# Autodesk Inventor assembly: Сборка
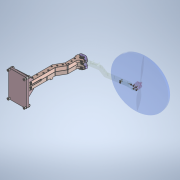
[picture p0: Inventor's stored thumbnail of the model, 180x180]
Saved by Autodesk Inventor 2021.2 (Build 252289000, 289)
## iProperties
Created: 2024-10-29
Part Number: Сборка
Document SubType Name: Assembly
Designer: barko
Mass: 1383.59 g
Surface Area: 2828.64 cm^2
Volume: 1218.78 cm^3
Density: 1.13522 g/cm^3
Author: barko
## Documents named in this file (33)
- C:\Users\DELL\Desktop\Personal\PID_controller\PID_controller\Mechanics\3D_model\Сборка.iam
- C:\Users\DELL\Desktop\Personal\PID_controller\PID_controller\Mechanics\3D_model\Детали твёрдого тела\Скобка 1.ipt
- C:\Users\DELL\Desktop\Personal\PID_controller\PID_controller\Mechanics\3D_model\Детали твёрдого тела\Скобка 2.ipt
- C:\Users\DELL\Desktop\Personal\PID_controller\PID_controller\Mechanics\3D_model\Детали твёрдого тела\Фланец.ipt
- C:\Users\DELL\Desktop\Personal\PID_controller\PID_controller\Mechanics\3D_model\Детали твёрдого тела\Луч.ipt
- C:\Users\DELL\Desktop\Personal\PID_controller\PID_controller\Mechanics\3D_model\Детали твёрдого тела\Ложечка.ipt
- C:\Users\DELL\Desktop\Personal\PID_controller\PID_controller\Mechanics\3D_model\Моторчик.ipt
- C:\Users\DELL\Desktop\Personal\PID_controller\PID_controller\Mechanics\3D_model\Пропеллер.ipt
- C:\Users\DELL\Documents\Inventor\Content Center Files\R2021\ru-RU\Nut GOST 15524-70\Гайка M4-6H ГОСТ 15524-70.ipt
- C:\Users\DELL\Documents\Inventor\Content Center Files\R2021\ru-RU\GOST 11738-84\Винт M4-6gx20 ГОСТ 11738-84.ipt
- C:\Users\DELL\Desktop\Personal\PID_controller\PID_controller\Mechanics\3D_model\Подшипник.ipt
- C:\Users\DELL\Documents\Inventor\Content Center Files\R2021\ru-RU\GOST 5915-70\Гайка M6-6H ГОСТ 5915-70(1).ipt
- C:\Users\DELL\Documents\Inventor\Content Center Files\R2021\ru-RU\GOST 11738-84\Винт M6-6gx50 ГОСТ 11738-84.ipt
- C:\Users\DELL\Documents\Inventor\Content Center Files\R2021\ru-RU\GOST 11371-78  A\Шайба 6 ГОСТ 11371-78.ipt
- C:\Users\DELL\Documents\Inventor\Content Center Files\R2021\ru-RU\Washer 1 GOST 6402-78\Шайба 6Л ГОСТ 6402-78.ipt
- C:\Users\DELL\Documents\Inventor\Content Center Files\R2021\ru-RU\GOST 17475-80 (2)\Винт 2.M6-6gx30 ГОСТ 17475-80.ipt
- C:\Users\DELL\Documents\Inventor\Content Center Files\R2021\ru-RU\ISO 10642(1)\ISO 10642 - M3x8.ipt
- C:\Users\DELL\Documents\Inventor\Content Center Files\R2021\ru-RU\ISO 10642(1)\ISO 10642 - M3x12.ipt
- C:\Users\DELL\Desktop\Personal\PID_controller\PID_controller\Mechanics\3D_model\Детали твёрдого тела\Вал насадка 1.ipt
- C:\Users\DELL\Desktop\Personal\PID_controller\PID_controller\Mechanics\3D_model\Метизы\Гайка M4-6H ГОСТ 11860-85.ipt
- C:\Users\DELL\Desktop\Personal\PID_controller\PID_controller\Mechanics\3D_model\Метизы\Шайба A 4 ГОСТ 6958-78.ipt
- C:\Users\DELL\Documents\Inventor\Content Center Files\R2021\ru-RU\GOST 5916-70\Гайка M4-6H ГОСТ 5916-70.ipt
- C:\Users\DELL\Documents\Inventor\Content Center Files\R2021\ru-RU\GOST 11738-84\Винт M4-6gx25 ГОСТ 11738-84.ipt
- C:\Users\DELL\Documents\Inventor\Content Center Files\R2021\ru-RU\GOST 11738-84\Винт M6-6gx30 ГОСТ 11738-84.ipt
- C:\Users\DELL\Desktop\Personal\PID_controller\PID_controller\Mechanics\3D_model\Детали твёрдого тела\Вал стержень.ipt
- C:\Users\DELL\Desktop\Personal\PID_controller\PID_controller\Mechanics\3D_model\Детали твёрдого тела\Блок.ipt
- C:\Users\DELL\Desktop\Personal\PID_controller\PID_controller\Mechanics\3D_model\Детали твёрдого тела\Ножка левая верх.ipt
- C:\Users\DELL\Desktop\Personal\PID_controller\PID_controller\Mechanics\3D_model\Детали твёрдого тела\Ножка левая низ.ipt
- C:\Users\DELL\Desktop\Personal\PID_controller\PID_controller\Mechanics\3D_model\Детали твёрдого тела\Ножка правая верх.ipt
- C:\Users\DELL\Desktop\Personal\PID_controller\PID_controller\Mechanics\3D_model\Детали твёрдого тела\Ножка правая низ.ipt
- C:\Users\DELL\Documents\Inventor\Content Center Files\R2021\ru-RU\GOST 11738-84\Винт M4-6gx30 ГОСТ 11738-84.ipt
- C:\Users\DELL\Desktop\Personal\PID_controller\PID_controller\Mechanics\3D_model\Метизы\Винт M3-6gx8 ГОСТ 11738-84.ipt
- C:\Users\DELL\Desktop\Personal\PID_controller\PID_controller\Mechanics\3D_model\Метизы\Винт M4-6gx40 ГОСТ 1491-80.ipt
## Components (83 placed, 32 different names)
1. Скобка 1:1 — Совмещение:104, Совмещение:109
2. Скобка 2:1 — Совмещение:119, Совмещение:120
3. Фланец:1 — Вставка:6, Вставка:7, Вставка:8, Вставка:9, Заподлицо:2, Заподлицо:3, Заподлицо:4, Заподлицо:5, Совмещение:127, Совмещение:128, Совмещение:129, Совмещение:130, Совмещение:131, Совмещение:132, Совмещение:133, Совмещение:134, Совмещение:135, Совмещение:136, Совмещение:137, Совмещение:138
4. Луч:1 — Заподлицо:1, Совмещение:96, Угол:2, Совмещение:97, Заподлицо:6, Совмещение:110, Совмещение:111, Совмещение:112, Совмещение:114, Совмещение:199
5. Ложечка:1 — Совмещение:87, Совмещение:88, Совмещение:91, Совмещение:92, Совмещение:93, Совмещение:94, Совмещение:96, Угол:2, Совмещение:97, Заподлицо:6, Совмещение:98, Совмещение:99, Вставка:37
6. Моторчик:1 — Вставка:2, Совмещение:98, Совмещение:99
7. Пропеллер:1 — Вставка:2
8. Подшипник:1 — Вставка:25, Вставка:29, Вставка:39
9. Подшипник:2 — Вставка:32, Вставка:34
10. Вал насадка 1:1 — Вставка:25, Вставка:32, Совмещение:125, Совмещение:199
11. Гайка M4-6H ГОСТ 11860-85:2
12. Шайба A 4 ГОСТ 6958-78:3 — Вставка:29, Вставка:33, Вставка:38
13. Вал стержень:1 — Совмещение:125, Заподлицо:7
14. Гайка ГОСТ 15524-70 M4:6 — Вставка:33, Заподлицо:7
15. Блок:1 — Вставка:35, Вставка:36, Совмещение:126
16. Шайба A 4 ГОСТ 6958-78:4 — Вставка:34, Вставка:35
17. Гайка ГОСТ 15524-70 M4:7 — Вставка:36, Совмещение:126
18. Ножка левая верх:1 — Совмещение:152, Совмещение:153, Совмещение:154, Совмещение:155, Совмещение:156, Совмещение:157, Совмещение:166, Совмещение:168, Совмещение:170, Совмещение:186, Совмещение:188, Совмещение:190, Совмещение:192, Совмещение:194, Совмещение:196, Совмещение:198
19. Ножка левая низ:1 — Совмещение:143, Совмещение:145
20. Ножка правая верх:1 — Совмещение:147, Совмещение:148, Совмещение:149, Совмещение:150, Совмещение:151, Совмещение:158, Совмещение:159, Совмещение:160, Совмещение:161, Совмещение:162, Совмещение:163, Совмещение:164, Совмещение:165, Совмещение:167, Совмещение:169, Вставка:39
21. Ножка правая низ:1 — Совмещение:144, Совмещение:146, Совмещение:171, Совмещение:172, Совмещение:173, Совмещение:174, Совмещение:175, Совмещение:176, Совмещение:177, Совмещение:178, Совмещение:179, Совмещение:180, Совмещение:181, Совмещение:182, Совмещение:183, Совмещение:184, Совмещение:185, Совмещение:187, Совмещение:189, Совмещение:191, Совмещение:193, Совмещение:195, Совмещение:197
22. Винт ГОСТ 11738-84 M 4x30:4 — Совмещение:171, Совмещение:172
23. Гайка ГОСТ 5916-70 M4:4 — Совмещение:185, Совмещение:186
24. Винт ГОСТ 11738-84 M 4x30:5 — Совмещение:173, Совмещение:174
25. Винт ГОСТ 11738-84 M 4x30:6 — Совмещение:175, Совмещение:176
26. Винт ГОСТ 11738-84 M 4x30:7 — Совмещение:177, Совмещение:178
27. Винт ГОСТ 11738-84 M 4x30:8 — Совмещение:179, Совмещение:180
28. Винт ГОСТ 11738-84 M 4x30:9 — Совмещение:181, Совмещение:182
29. Винт ГОСТ 11738-84 M 4x30:10 — Совмещение:183, Совмещение:184
30. Гайка ГОСТ 5916-70 M4:5 — Совмещение:187, Совмещение:188
31. Гайка ГОСТ 5916-70 M4:6 — Совмещение:189, Совмещение:190
32. Гайка ГОСТ 5916-70 M4:7 — Совмещение:191, Совмещение:192
33. Гайка ГОСТ 5916-70 M4:8 — Совмещение:193, Совмещение:194
34. Гайка ГОСТ 5916-70 M4:9 — Совмещение:195, Совмещение:196
35. Гайка ГОСТ 5916-70 M4:10 — Совмещение:197, Совмещение:198
36. Винт M3-6gx8 ГОСТ 11738-84:1 — Вставка:37
37. Винт M4-6gx40 ГОСТ 1491-80:1 — Вставка:38
38. Гайка ГОСТ 5916-70 M4:3 — Совмещение:169, Совмещение:170
39. Гайка ГОСТ 5916-70 M4:2 — Совмещение:167, Совмещение:168
40. Винт ГОСТ 11738-84 M 4x30:3 — Совмещение:163, Совмещение:164
41. Винт ГОСТ 11738-84 M 4x30:2 — Совмещение:161, Совмещение:162
42. Гайка ГОСТ 5916-70 M4:1 — Совмещение:165, Совмещение:166
43. Винт ГОСТ 11738-84 M 4x30:1 — Совмещение:159, Совмещение:160
44. Винт ГОСТ 11738-84 M 4x25:1 — Совмещение:103, Совмещение:104
45. Гайка ГОСТ 15524-70 M4:1 — Совмещение:103, Совмещение:147, Совмещение:148, Совмещение:149
46. Винт ГОСТ 11738-84 M 4x25:2 — Совмещение:113, Совмещение:114
47. Гайка ГОСТ 15524-70 M4:2 — Совмещение:110, Совмещение:111, Совмещение:112, Совмещение:113
48. Винт ГОСТ 11738-84 M 4x20:2 — Совмещение:108, Совмещение:109
49. Винт ГОСТ 11738-84 M 4x25:3 — Совмещение:118, Совмещение:119
50. Винт ГОСТ 11738-84 M 4x20:4 — Совмещение:120, Совмещение:124
51. Гайка ГОСТ 15524-70 M4:3 — Совмещение:118, Совмещение:155, Совмещение:156, Совмещение:157
52. Гайка ГОСТ 15524-70 M4:4 — Совмещение:108, Совмещение:150, Совмещение:151, Совмещение:158
53. Гайка ГОСТ 15524-70 M4:5 — Совмещение:124, Совмещение:152, Совмещение:153, Совмещение:154
54. Гайка ГОСТ 5915-70 M6:1 — Совмещение:133, Совмещение:134, Совмещение:135, Совмещение:140
55. Гайка ГОСТ 5915-70 M6:2 — Совмещение:127, Совмещение:128, Совмещение:129, Совмещение:139
56. Гайка ГОСТ 5915-70 M6:3 — Совмещение:136, Совмещение:137, Совмещение:138, Совмещение:141
57. Гайка ГОСТ 5915-70 M6:4 — Совмещение:78, Совмещение:130, Совмещение:131, Совмещение:132, Совмещение:142
58. Винт ГОСТ 11738-84 M 6x50:1 — Совмещение:141, Совмещение:146
59. Винт ГОСТ 11738-84 M 6x30:1 — Совмещение:139, Совмещение:143
60. Винт ГОСТ 11738-84 M 6x30:2 — Совмещение:78, Совмещение:142, Совмещение:144
61. Винт ГОСТ 11738-84 M 6x50:2 — Совмещение:140, Совмещение:145
62. Шайба  ГОСТ 11371-78 6,4:1 — Вставка:6, Вставка:10
63. Шайба  ГОСТ 11371-78 6,4:2 — Вставка:7, Вставка:11
64. Шайба  ГОСТ 11371-78 6,4:3 — Вставка:8, Вставка:13
65. Шайба  ГОСТ 11371-78 6,4:4 — Вставка:9, Вставка:12
66. Шайба 1 ГОСТ 6402-78 6Л:1 — Вставка:10, Вставка:16
67. Шайба 1 ГОСТ 6402-78 6Л:2 — Вставка:11, Вставка:15
68. Шайба 1 ГОСТ 6402-78 6Л:3 — Вставка:12, Вставка:17
69. Шайба 1 ГОСТ 6402-78 6Л:4 — Вставка:13, Вставка:14
70. Гайка ГОСТ 5915-70 M6:5 — Вставка:14, Совмещение:85
71. Гайка ГОСТ 5915-70 M6:6 — Вставка:15, Совмещение:84
72. Гайка ГОСТ 5915-70 M6:7 — Вставка:16, Совмещение:82
73. Гайка ГОСТ 5915-70 M6:8 — Вставка:17, Совмещение:83
74. Винт 2 ГОСТ 17475-80 M6 x 30:1 — Совмещение:82, Заподлицо:3
75. Винт 2 ГОСТ 17475-80 M6 x 30:2 — Совмещение:83, Заподлицо:2
76. Винт 2 ГОСТ 17475-80 M6 x 30:3 — Совмещение:85, Заподлицо:5
77. Винт 2 ГОСТ 17475-80 M6 x 30:4 — Совмещение:84, Заподлицо:4
78. ISO 10642 M3x12:2 — Совмещение:87
79. ISO 10642 M3x12:3 — Совмещение:88
80. ISO 10642 M3x8:1 — Совмещение:91
81. ISO 10642 M3x8:2 — Совмещение:92
82. ISO 10642 M3x8:3 — Совмещение:93
83. ISO 10642 M3x8:4 — Совмещение:94
## Relationships (134: Mate 103, Insert 23, Flush 7, Angle 1)
- Вставка:2 [Insert] (2 mm): Моторчик:1 ↔ Пропеллер:1
- Заподлицо:1 [Flush]: Луч:1
- Совмещение:78 [Mate]: Гайка ГОСТ 5915-70 M6:4 ↔ Винт ГОСТ 11738-84 M 6x30:2
- Вставка:6 [Insert]: Фланец:1 ↔ Шайба  ГОСТ 11371-78 6,4:1
- Вставка:7 [Insert]: Фланец:1 ↔ Шайба  ГОСТ 11371-78 6,4:2
- Вставка:8 [Insert]: Фланец:1 ↔ Шайба  ГОСТ 11371-78 6,4:3
- Вставка:9 [Insert]: Фланец:1 ↔ Шайба  ГОСТ 11371-78 6,4:4
- Вставка:10 [Insert]: Шайба  ГОСТ 11371-78 6,4:1 ↔ Шайба 1 ГОСТ 6402-78 6Л:1
- Вставка:11 [Insert]: Шайба  ГОСТ 11371-78 6,4:2 ↔ Шайба 1 ГОСТ 6402-78 6Л:2
- Вставка:12 [Insert]: Шайба  ГОСТ 11371-78 6,4:4 ↔ Шайба 1 ГОСТ 6402-78 6Л:3
- Вставка:13 [Insert]: Шайба  ГОСТ 11371-78 6,4:3 ↔ Шайба 1 ГОСТ 6402-78 6Л:4
- Вставка:14 [Insert]: Шайба 1 ГОСТ 6402-78 6Л:4 ↔ Гайка ГОСТ 5915-70 M6:5
- Вставка:15 [Insert]: Шайба 1 ГОСТ 6402-78 6Л:2 ↔ Гайка ГОСТ 5915-70 M6:6
- Вставка:16 [Insert]: Шайба 1 ГОСТ 6402-78 6Л:1 ↔ Гайка ГОСТ 5915-70 M6:7
- Вставка:17 [Insert]: Шайба 1 ГОСТ 6402-78 6Л:3 ↔ Гайка ГОСТ 5915-70 M6:8
- Совмещение:82 [Mate]: Гайка ГОСТ 5915-70 M6:7 ↔ Винт 2 ГОСТ 17475-80 M6 x 30:1
- Совмещение:83 [Mate]: Гайка ГОСТ 5915-70 M6:8 ↔ Винт 2 ГОСТ 17475-80 M6 x 30:2
- Совмещение:84 [Mate]: Гайка ГОСТ 5915-70 M6:6 ↔ Винт 2 ГОСТ 17475-80 M6 x 30:4
- Совмещение:85 [Mate]: Гайка ГОСТ 5915-70 M6:5 ↔ Винт 2 ГОСТ 17475-80 M6 x 30:3
- Заподлицо:2 [Flush] (9 mm): Фланец:1 ↔ Винт 2 ГОСТ 17475-80 M6 x 30:2
- Заподлицо:3 [Flush] (9 mm): Фланец:1 ↔ Винт 2 ГОСТ 17475-80 M6 x 30:1
- Заподлицо:4 [Flush] (9 mm): Фланец:1 ↔ Винт 2 ГОСТ 17475-80 M6 x 30:4
- Заподлицо:5 [Flush] (9 mm): Фланец:1 ↔ Винт 2 ГОСТ 17475-80 M6 x 30:3
- Совмещение:87 [Mate]: Ложечка:1 ↔ ISO 10642 M3x12:2
- Совмещение:88 [Mate]: Ложечка:1 ↔ ISO 10642 M3x12:3
- Совмещение:91 [Mate]: Ложечка:1 ↔ ISO 10642 M3x8:1
- Совмещение:92 [Mate]: Ложечка:1 ↔ ISO 10642 M3x8:2
- Совмещение:93 [Mate]: Ложечка:1 ↔ ISO 10642 M3x8:3
- Совмещение:94 [Mate]: Ложечка:1 ↔ ISO 10642 M3x8:4
- Совмещение:96 [Mate]: Луч:1 ↔ Ложечка:1
- Угол:2 [Angle] (180 deg): Луч:1 ↔ Ложечка:1
- Совмещение:97 [Mate]: Луч:1 ↔ Ложечка:1
- Заподлицо:6 [Flush]: Луч:1 ↔ Ложечка:1
- Совмещение:98 [Mate]: Ложечка:1 ↔ Моторчик:1
- Совмещение:99 [Mate]: Ложечка:1 ↔ Моторчик:1
- Вставка:25 [Insert]: Подшипник:1 ↔ Вал насадка 1:1
- Совмещение:103 [Mate]: Винт ГОСТ 11738-84 M 4x25:1 ↔ Гайка ГОСТ 15524-70 M4:1
- Совмещение:104 [Mate]: Скобка 1:1 ↔ Винт ГОСТ 11738-84 M 4x25:1
- Совмещение:108 [Mate]: Винт ГОСТ 11738-84 M 4x20:2 ↔ Гайка ГОСТ 15524-70 M4:4
- Совмещение:109 [Mate]: Скобка 1:1 ↔ Винт ГОСТ 11738-84 M 4x20:2
- Совмещение:110 [Mate]: Луч:1 ↔ Гайка ГОСТ 15524-70 M4:2
- Совмещение:111 [Mate]: Луч:1 ↔ Гайка ГОСТ 15524-70 M4:2
- Совмещение:112 [Mate]: Луч:1 ↔ Гайка ГОСТ 15524-70 M4:2
- Совмещение:113 [Mate]: Винт ГОСТ 11738-84 M 4x25:2 ↔ Гайка ГОСТ 15524-70 M4:2
- Совмещение:114 [Mate]: Луч:1 ↔ Винт ГОСТ 11738-84 M 4x25:2
- Совмещение:118 [Mate]: Винт ГОСТ 11738-84 M 4x25:3 ↔ Гайка ГОСТ 15524-70 M4:3
- Совмещение:119 [Mate]: Скобка 2:1 ↔ Винт ГОСТ 11738-84 M 4x25:3
- Совмещение:120 [Mate]: Скобка 2:1 ↔ Винт ГОСТ 11738-84 M 4x20:4
- Совмещение:124 [Mate]: Винт ГОСТ 11738-84 M 4x20:4 ↔ Гайка ГОСТ 15524-70 M4:5
- Вставка:29 [Insert]: Подшипник:1 ↔ Шайба A 4 ГОСТ 6958-78:3
- Вставка:32 [Insert]: Подшипник:2 ↔ Вал насадка 1:1
- Совмещение:125 [Mate]: Вал насадка 1:1 ↔ Вал стержень:1
- Вставка:33 [Insert]: Шайба A 4 ГОСТ 6958-78:3 ↔ Гайка ГОСТ 15524-70 M4:6
- Заподлицо:7 [Flush] (-2 mm): Вал стержень:1 ↔ Гайка ГОСТ 15524-70 M4:6
- Вставка:34 [Insert]: Подшипник:2 ↔ Шайба A 4 ГОСТ 6958-78:4
- Вставка:35 [Insert]: Блок:1 ↔ Шайба A 4 ГОСТ 6958-78:4
- Вставка:36 [Insert]: Блок:1 ↔ Гайка ГОСТ 15524-70 M4:7
- Совмещение:126 [Mate]: Блок:1 ↔ Гайка ГОСТ 15524-70 M4:7
- Совмещение:127 [Mate]: Фланец:1 ↔ Гайка ГОСТ 5915-70 M6:2
- Совмещение:128 [Mate]: Фланец:1 ↔ Гайка ГОСТ 5915-70 M6:2
- Совмещение:129 [Mate]: Фланец:1 ↔ Гайка ГОСТ 5915-70 M6:2
- Совмещение:130 [Mate]: Фланец:1 ↔ Гайка ГОСТ 5915-70 M6:4
- Совмещение:131 [Mate]: Фланец:1 ↔ Гайка ГОСТ 5915-70 M6:4
- Совмещение:132 [Mate]: Фланец:1 ↔ Гайка ГОСТ 5915-70 M6:4
- Совмещение:133 [Mate]: Фланец:1 ↔ Гайка ГОСТ 5915-70 M6:1
- Совмещение:134 [Mate]: Фланец:1 ↔ Гайка ГОСТ 5915-70 M6:1
- Совмещение:135 [Mate]: Фланец:1 ↔ Гайка ГОСТ 5915-70 M6:1
- Совмещение:136 [Mate]: Фланец:1 ↔ Гайка ГОСТ 5915-70 M6:3
- Совмещение:137 [Mate]: Фланец:1 ↔ Гайка ГОСТ 5915-70 M6:3
- Совмещение:138 [Mate]: Фланец:1 ↔ Гайка ГОСТ 5915-70 M6:3
- Совмещение:139 [Mate]: Гайка ГОСТ 5915-70 M6:2 ↔ Винт ГОСТ 11738-84 M 6x30:1
- Совмещение:140 [Mate]: Гайка ГОСТ 5915-70 M6:1 ↔ Винт ГОСТ 11738-84 M 6x50:2
- Совмещение:141 [Mate]: Гайка ГОСТ 5915-70 M6:3 ↔ Винт ГОСТ 11738-84 M 6x50:1
- Совмещение:142 [Mate]: Гайка ГОСТ 5915-70 M6:4 ↔ Винт ГОСТ 11738-84 M 6x30:2
- Совмещение:143 [Mate]: Ножка левая низ:1 ↔ Винт ГОСТ 11738-84 M 6x30:1
- Совмещение:144 [Mate]: Ножка правая низ:1 ↔ Винт ГОСТ 11738-84 M 6x30:2
- Совмещение:145 [Mate]: Ножка левая низ:1 ↔ Винт ГОСТ 11738-84 M 6x50:2
- Совмещение:146 [Mate]: Ножка правая низ:1 ↔ Винт ГОСТ 11738-84 M 6x50:1
- Совмещение:147 [Mate]: Ножка правая верх:1 ↔ Гайка ГОСТ 15524-70 M4:1
- Совмещение:148 [Mate]: Ножка правая верх:1 ↔ Гайка ГОСТ 15524-70 M4:1
- Совмещение:149 [Mate]: Ножка правая верх:1 ↔ Гайка ГОСТ 15524-70 M4:1
- Совмещение:150 [Mate]: Ножка правая верх:1 ↔ Гайка ГОСТ 15524-70 M4:4
- Совмещение:151 [Mate]: Ножка правая верх:1 ↔ Гайка ГОСТ 15524-70 M4:4
- Совмещение:152 [Mate]: Ножка левая верх:1 ↔ Гайка ГОСТ 15524-70 M4:5
- Совмещение:153 [Mate]: Ножка левая верх:1 ↔ Гайка ГОСТ 15524-70 M4:5
- Совмещение:154 [Mate]: Ножка левая верх:1 ↔ Гайка ГОСТ 15524-70 M4:5
- Совмещение:155 [Mate]: Ножка левая верх:1 ↔ Гайка ГОСТ 15524-70 M4:3
- Совмещение:156 [Mate]: Ножка левая верх:1 ↔ Гайка ГОСТ 15524-70 M4:3
- Совмещение:157 [Mate]: Ножка левая верх:1 ↔ Гайка ГОСТ 15524-70 M4:3
- Совмещение:158 [Mate]: Ножка правая верх:1 ↔ Гайка ГОСТ 15524-70 M4:4
- Совмещение:159 [Mate]: Ножка правая верх:1 ↔ Винт ГОСТ 11738-84 M 4x30:1
- Совмещение:160 [Mate]: Ножка правая верх:1 ↔ Винт ГОСТ 11738-84 M 4x30:1
- Совмещение:161 [Mate]: Ножка правая верх:1 ↔ Винт ГОСТ 11738-84 M 4x30:2
- Совмещение:162 [Mate]: Ножка правая верх:1 ↔ Винт ГОСТ 11738-84 M 4x30:2
- Совмещение:163 [Mate]: Ножка правая верх:1 ↔ Винт ГОСТ 11738-84 M 4x30:3
- Совмещение:164 [Mate]: Ножка правая верх:1 ↔ Винт ГОСТ 11738-84 M 4x30:3
- Совмещение:165 [Mate]: Ножка правая верх:1 ↔ Гайка ГОСТ 5916-70 M4:1
- Совмещение:166 [Mate]: Ножка левая верх:1 ↔ Гайка ГОСТ 5916-70 M4:1
- Совмещение:167 [Mate]: Ножка правая верх:1 ↔ Гайка ГОСТ 5916-70 M4:2
- Совмещение:168 [Mate]: Ножка левая верх:1 ↔ Гайка ГОСТ 5916-70 M4:2
- Совмещение:169 [Mate]: Ножка правая верх:1 ↔ Гайка ГОСТ 5916-70 M4:3
- Совмещение:170 [Mate]: Ножка левая верх:1 ↔ Гайка ГОСТ 5916-70 M4:3
- Совмещение:171 [Mate]: Ножка правая низ:1 ↔ Винт ГОСТ 11738-84 M 4x30:4
- Совмещение:172 [Mate]: Ножка правая низ:1 ↔ Винт ГОСТ 11738-84 M 4x30:4
- Совмещение:173 [Mate]: Ножка правая низ:1 ↔ Винт ГОСТ 11738-84 M 4x30:5
- Совмещение:174 [Mate]: Ножка правая низ:1 ↔ Винт ГОСТ 11738-84 M 4x30:5
- Совмещение:175 [Mate]: Ножка правая низ:1 ↔ Винт ГОСТ 11738-84 M 4x30:6
- Совмещение:176 [Mate]: Ножка правая низ:1 ↔ Винт ГОСТ 11738-84 M 4x30:6
- Совмещение:177 [Mate]: Ножка правая низ:1 ↔ Винт ГОСТ 11738-84 M 4x30:7
- Совмещение:178 [Mate]: Ножка правая низ:1 ↔ Винт ГОСТ 11738-84 M 4x30:7
- Совмещение:179 [Mate]: Ножка правая низ:1 ↔ Винт ГОСТ 11738-84 M 4x30:8
- Совмещение:180 [Mate]: Ножка правая низ:1 ↔ Винт ГОСТ 11738-84 M 4x30:8
- Совмещение:181 [Mate]: Ножка правая низ:1 ↔ Винт ГОСТ 11738-84 M 4x30:9
- Совмещение:182 [Mate]: Ножка правая низ:1 ↔ Винт ГОСТ 11738-84 M 4x30:9
- Совмещение:183 [Mate]: Ножка правая низ:1 ↔ Винт ГОСТ 11738-84 M 4x30:10
- Совмещение:184 [Mate]: Ножка правая низ:1 ↔ Винт ГОСТ 11738-84 M 4x30:10
- Совмещение:185 [Mate]: Ножка правая низ:1 ↔ Гайка ГОСТ 5916-70 M4:4
- Совмещение:186 [Mate]: Ножка левая верх:1 ↔ Гайка ГОСТ 5916-70 M4:4
- Совмещение:187 [Mate]: Ножка правая низ:1 ↔ Гайка ГОСТ 5916-70 M4:5
- Совмещение:188 [Mate]: Ножка левая верх:1 ↔ Гайка ГОСТ 5916-70 M4:5
- Совмещение:189 [Mate]: Ножка правая низ:1 ↔ Гайка ГОСТ 5916-70 M4:6
- Совмещение:190 [Mate]: Ножка левая верх:1 ↔ Гайка ГОСТ 5916-70 M4:6
- Совмещение:191 [Mate]: Ножка правая низ:1 ↔ Гайка ГОСТ 5916-70 M4:7
- Совмещение:192 [Mate]: Ножка левая верх:1 ↔ Гайка ГОСТ 5916-70 M4:7
- Совмещение:193 [Mate]: Ножка правая низ:1 ↔ Гайка ГОСТ 5916-70 M4:8
- Совмещение:194 [Mate]: Ножка левая верх:1 ↔ Гайка ГОСТ 5916-70 M4:8
- Совмещение:195 [Mate]: Ножка правая низ:1 ↔ Гайка ГОСТ 5916-70 M4:9
- Совмещение:196 [Mate]: Ножка левая верх:1 ↔ Гайка ГОСТ 5916-70 M4:9
- Совмещение:197 [Mate]: Ножка правая низ:1 ↔ Гайка ГОСТ 5916-70 M4:10
- Совмещение:198 [Mate]: Ножка левая верх:1 ↔ Гайка ГОСТ 5916-70 M4:10
- Вставка:37 [Insert]: Ложечка:1 ↔ Винт M3-6gx8 ГОСТ 11738-84:1
- Вставка:38 [Insert]: Шайба A 4 ГОСТ 6958-78:3 ↔ Винт M4-6gx40 ГОСТ 1491-80:1
- Вставка:39 [Insert]: Подшипник:1 ↔ Ножка правая верх:1
- Совмещение:199 [Mate]: Луч:1 ↔ Вал насадка 1:1
